# Autodesk Inventor assembly: AM14U3 Square Half
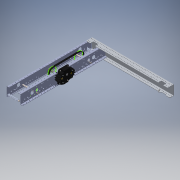
[picture p0: Inventor's stored thumbnail of the model, 180x180]
Saved by Autodesk Inventor 2016 (Build 200138000, 138)
## iProperties
Created: 2016-01-27
Part Number: AM14U3 Square Half
Document SubType Name: Assembly
Designer: PrashantBIA
Author: PrashantBIA
Revision Number: ANY
## Documents named in this file (7)
- C:\Users\GEH-Magnet School 1\Documents\GitHub\2016RobotCADFiles\Drive Train\AM14U3 Square Half.iam
- C:\Users\GEH-Magnet School 1\Documents\GitHub\2016RobotCADFiles\Drive Train\AM14U3 Square Frame Half.iam
- C:\Users\GEH-Magnet School 1\Documents\GitHub\2016RobotCADFiles\Drive Train\am-2598_107 2016 KOP Toughbox Mini.iam
- C:\Users\GEH-Magnet School 1\Documents\GitHub\2016RobotCADFiles\Drive Train\FR8ZZ Hex Bearing.ipt
- C:\Users\GEH-Magnet School 1\Documents\GitHub\2016RobotCADFiles\Drive Train\375-16 x 4.25 Hex Bolt_HFBOLT 0.375-16x2.5x1-C.ipt
- C:\Users\GEH-Magnet School 1\Documents\GitHub\2016RobotCADFiles\Drive Train\375-16 Lock Nut_91831A127.ipt
- C:\Users\GEH-Magnet School 1\Documents\GitHub\2016RobotCADFiles\Drive Train\am-2571 655-5M-15 Timing Belt.ipt
## Components (8 placed, 8 different names)
1. AM14U3 Square Frame Half_3 [sub-assembly] — Mate:1, Mate:2, Mate:3, Mate:4, Mate:7, Mate:8, Mate:9, Mate:10, Mate:12, Mate:13
2. am-2598_107 2016 KOP Toughbox Mini_4 [sub-assembly] — Mate:1, Mate:2, Mate:3
3. FR8ZZ Hex Bearing_8 — Mate:7, Mate:8, Mate:15
4. 375-16 x 4.25 Hex Bolt_HFBOLT 0.375-16x2.5x1-C_9 — Mate:12, Mate:13, Mate:14
5. 375-16 x 4.25 Hex Bolt_HFBOLT 0.375-16x2.5x1-C_10 — Mate:9, Mate:10, Mate:11
6. 375-16 Lock Nut_91831A127_12
7. am-2571 655-5M-15 Timing Belt_13 — Mate:4, Mate:14, Mate:15
8. am-2571 655-5M-15 Timing Belt_14 — Mate:11
## Relationships (13: Mate 13)
- Mate:1: AM14U3 Square Frame Half_3 ↔ am-2598_107 2016 KOP Toughbox Mini_4
- Mate:2: AM14U3 Square Frame Half_3 ↔ am-2598_107 2016 KOP Toughbox Mini_4
- Mate:3: AM14U3 Square Frame Half_3 ↔ am-2598_107 2016 KOP Toughbox Mini_4
- Mate:4 (12.7 mm): AM14U3 Square Frame Half_3 ↔ am-2571 655-5M-15 Timing Belt_13
- Mate:7: AM14U3 Square Frame Half_3 ↔ FR8ZZ Hex Bearing_8
- Mate:8: AM14U3 Square Frame Half_3 ↔ FR8ZZ Hex Bearing_8
- Mate:9: AM14U3 Square Frame Half_3 ↔ 375-16 x 4.25 Hex Bolt_HFBOLT 0.375-16x2.5x1-C_10
- Mate:10: AM14U3 Square Frame Half_3 ↔ 375-16 x 4.25 Hex Bolt_HFBOLT 0.375-16x2.5x1-C_10
- Mate:11: 375-16 x 4.25 Hex Bolt_HFBOLT 0.375-16x2.5x1-C_10 ↔ am-2571 655-5M-15 Timing Belt_14
- Mate:12: AM14U3 Square Frame Half_3 ↔ 375-16 x 4.25 Hex Bolt_HFBOLT 0.375-16x2.5x1-C_9
- Mate:13: AM14U3 Square Frame Half_3 ↔ 375-16 x 4.25 Hex Bolt_HFBOLT 0.375-16x2.5x1-C_9
- Mate:14: 375-16 x 4.25 Hex Bolt_HFBOLT 0.375-16x2.5x1-C_9 ↔ am-2571 655-5M-15 Timing Belt_13
- Mate:15: FR8ZZ Hex Bearing_8 ↔ am-2571 655-5M-15 Timing Belt_13
